# Autodesk Inventor assembly: NM.PMTController.LightInterlock.Box
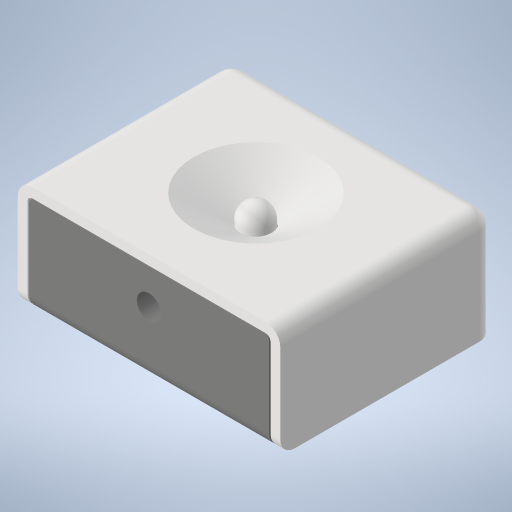
[picture p0: Inventor's stored thumbnail of the model, 512x512]
Saved by Autodesk Inventor 2023 (Build 270158000, 158)
## iProperties
Created: 2023-09-26
Part Number: NM.PMTController.LightInterlock.Box
Document SubType Name: Assembly
Designer: Graeme
Author: Graeme
## Documents named in this file (4)
- C:\Work\Inventor\Projects\test\mCAD\DualPMTController.LightInterlock.Box.iam
- C:\Work\Inventor\Projects\_PMTController\mCAD\NM.PMTController.LightInterlock\DualPMTController.LightInterlock.Top.ipt
- C:\Work\Inventor\Projects\_PMTController\mCAD\NM.PMTController.LightInterlock\DualPMTController.LightInterlock.Bottom.ipt
- C:\Work\Inventor\Projects\test\mCAD\Light Interlock\Dual PMT Controller - Light Interlock.iam
## Components (3 placed, 3 different names)
1. DualPMTController.LightInterlock.Top:1
2. DualPMTController.LightInterlock.Bottom:1 — Mate:1, Mate:2, Mate:3
3. Dual PMT Controller - Light Interlock:1 [sub-assembly] — Mate:1, Mate:2, Mate:3
## Relationships (3: Mate 3)
- Mate:1: DualPMTController.LightInterlock.Bottom:1 ↔ Dual PMT Controller - Light Interlock:1
- Mate:2: DualPMTController.LightInterlock.Bottom:1 ↔ Dual PMT Controller - Light Interlock:1
- Mate:3: DualPMTController.LightInterlock.Bottom:1 ↔ Dual PMT Controller - Light Interlock:1
